# Autodesk Inventor assembly: 08-03-00-000_shifter_assembly
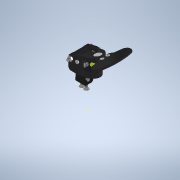
[picture p0: Inventor's stored thumbnail of the model, 180x180]
Saved by Autodesk Inventor 2020 (Build 240168000, 168)
## iProperties
Created: 2021-05-29
Part Number: 08-03-00-000_shifter_assembly
Document SubType Name: Assembly
Designer: Eric
Mass: 132.863 g
Surface Area: 203.28 cm^2
Volume: 20.5558 cm^3
Density: 6.46353 g/cm^3
Author: Eric
## Documents named in this file (15)
- C:\Users\Eric\Documents\repos\DIY_CAD_WheelButtonPlate\CAD\Inventor\08-05-00-000_shifter_assembly.iam
- C:\Users\Eric\Documents\repos\DIY_CAD_WheelButtonPlate\CAD\Inventor\08-05-01-002_shifter_base.ipt
- C:\Users\Eric\Documents\repos\DIY_CAD_WheelButtonPlate\CAD\Inventor\08-05-01-004_shifter_bottom.ipt
- C:\Users\Eric\Documents\repos\DIY_CAD_WheelButtonPlate\CAD\Inventor\08-05-01-003_shift_lever.ipt
- C:\Users\Eric\Documents\Inventor\Content Center Files\R2020\de-DE\DIN 7984\DIN 7984 - M3 x 8.ipt
- C:\Users\Eric\Documents\Inventor\Content Center Files\R2020\de-DE\DIN 7991(2)\DIN 7991 - M3x10.ipt
- C:\Users\Eric\Documents\Inventor\Content Center Files\R2020\de-DE\ISO 4035(1)\ISO 4035 - M3DIN EN.ipt
- C:\Users\Eric\Documents\repos\DIY_CAD_WheelButtonPlate\CAD\Inventor\08-05-01-005_shiftAndClutchHolder.ipt
- C:\Users\Eric\Documents\Inventor\Content Center Files\R2020\de-DE\DIN 7991(2)\DIN 7991 - M4x16.ipt
- C:\Users\Eric\Documents\Inventor\Content Center Files\R2020\de-DE\ISO 4032(1)\ISO 4032 - M4DIN EN.ipt
- C:\Users\Eric\Documents\repos\DIY_CAD_WheelButtonPlate\CAD\Inventor\08-05-02-006_Apem_yellow.ipt
- C:\Users\Eric\Documents\Inventor\Content Center Files\R2020\de-DE\ISO 4762(1)\DIN EN ISO 4762 - M4 x 40.ipt
- C:\Users\Eric\Documents\Inventor\Content Center Files\R2020\de-DE\ISO 4032(1)\ISO 4032 - M3DIN EN.ipt
- C:\Users\Eric\Documents\repos\DIY_CAD_WheelButtonPlate\CAD\Inventor\08-05-01-001_shifter_paddle.ipt
- C:\Users\Eric\Documents\repos\DIY_CAD_WheelButtonPlate\CAD\Inventor\08-04-02-004_magnet12x3.ipt
## Components (26 placed, 14 different names)
1. 08-05-01-002_shifter_base — Passend:5, Passend:16, Passend:17, Passend:18, Passend:26, Passend:27, Passend:29, Passend:31, Einfügen:5, Einfügen:6, Einfügen:9, Einfügen:10, Winkel:2, Winkel:3, Passend:38
2. 08-05-01-004_shifter_bottom — Passend:5, Passend:8, Winkel:1, Einfügen:7, Einfügen:8, Passend:36, Passend:37, Passend:39, Passend:40
3. 08-05-01-003_shift_lever — Passend:8, Passend:10, Passend:11, Fluchtend:2, Passend:13, Passend:15, Winkel:1, Passend:32, Passend:35, Passend:41, Passend:42
4. DIN 7984 M3 x 8:1 — Passend:31
5. DIN 7984 M3 x 8:2 — Passend:29, Passend:37, Passend:38
6. DIN 7991 M3x10:1 — Passend:11, Fluchtend:1, Fluchtend:2, Passend:12, Passend:34
7. DIN 7991 M3x10:2 — Passend:10, Fluchtend:1, Passend:14, Passend:33
8. DIN EN 24035 M3:1 — Passend:12, Passend:13
9. DIN EN 24035 M3:2 — Passend:14, Passend:15
10. 08-05-01-005_shiftAndClutchHolder:1 — Passend:16, Passend:17, Passend:18, Passend:19, Passend:20, Passend:21, Passend:22, Passend:23, Einfügen:3, Einfügen:4, Passend:24, Passend:25
11. DIN 7991 M4x16:1 — Passend:19
12. DIN 7991 M4x16:2 — Passend:20
13. DIN 7991 M4x16:3 — Passend:22, Fluchtend:3
14. DIN 7991 M4x16:4 — Passend:21, Fluchtend:3, Passend:23
15. DIN EN 24032 M4:1 — Einfügen:3, Passend:24
16. DIN EN 24032 M4:2 — Einfügen:4, Passend:25
17. 08-05-02-006_Apem_yellow:1 — Passend:26, Passend:27
18. DIN EN ISO 4762 M4 x 40:1 — Einfügen:5, Passend:35, Passend:36
19. DIN EN 24032 M4:3 — Einfügen:6
20. DIN EN 24032 M3:1 — Einfügen:7
21. DIN EN 24032 M3:2 — Einfügen:8
22. 08-05-01-001_shifter_paddle:1 — Passend:32, Passend:33, Passend:34
23. DIN EN 24032 M4:4 — Einfügen:9, Winkel:2
24. DIN EN 24032 M4:5 — Einfügen:10, Winkel:3
25. 08-04-02-004_magnet12x3:1 — Passend:39, Passend:40
26. 08-04-02-004_magnet12x3:2 — Passend:41, Passend:42
## Relationships (47: Mate 33, Insert 8, Flush 3, Angle 3)
- Passend:5 [Mate] (0.4 mm): 08-05-01-002_shifter_base ↔ 08-05-01-004_shifter_bottom
- Passend:8 [Mate] (0.2 mm): 08-05-01-004_shifter_bottom ↔ 08-05-01-003_shift_lever
- Passend:10 [Mate]: 08-05-01-003_shift_lever ↔ DIN 7991 M3x10:2
- Passend:11 [Mate]: 08-05-01-003_shift_lever ↔ DIN 7991 M3x10:1
- Fluchtend:1 [Flush]: DIN 7991 M3x10:1 ↔ DIN 7991 M3x10:2
- Fluchtend:2 [Flush] (-3.1 mm): 08-05-01-003_shift_lever ↔ DIN 7991 M3x10:1
- Passend:12 [Mate]: DIN 7991 M3x10:1 ↔ DIN EN 24035 M3:1
- Passend:13 [Mate]: 08-05-01-003_shift_lever ↔ DIN EN 24035 M3:1
- Passend:14 [Mate]: DIN 7991 M3x10:2 ↔ DIN EN 24035 M3:2
- Passend:15 [Mate]: 08-05-01-003_shift_lever ↔ DIN EN 24035 M3:2
- Passend:16 [Mate] (2 mm): 08-05-01-002_shifter_base ↔ 08-05-01-005_shiftAndClutchHolder:1
- Passend:17 [Mate]: 08-05-01-002_shifter_base ↔ 08-05-01-005_shiftAndClutchHolder:1
- Passend:18 [Mate]: 08-05-01-002_shifter_base ↔ 08-05-01-005_shiftAndClutchHolder:1
- Winkel:1 [Angle] (180 deg): 08-05-01-004_shifter_bottom ↔ 08-05-01-003_shift_lever
- Passend:19 [Mate]: 08-05-01-005_shiftAndClutchHolder:1 ↔ DIN 7991 M4x16:1
- Passend:20 [Mate]: 08-05-01-005_shiftAndClutchHolder:1 ↔ DIN 7991 M4x16:2
- Passend:21 [Mate]: 08-05-01-005_shiftAndClutchHolder:1 ↔ DIN 7991 M4x16:4
- Passend:22 [Mate]: 08-05-01-005_shiftAndClutchHolder:1 ↔ DIN 7991 M4x16:3
- Fluchtend:3 [Flush]: DIN 7991 M4x16:3 ↔ DIN 7991 M4x16:4
- Passend:23 [Mate] (-16.1 mm): 08-05-01-005_shiftAndClutchHolder:1 ↔ DIN 7991 M4x16:4
- Einfügen:3 [Insert]: 08-05-01-005_shiftAndClutchHolder:1 ↔ DIN EN 24032 M4:1
- Einfügen:4 [Insert]: 08-05-01-005_shiftAndClutchHolder:1 ↔ DIN EN 24032 M4:2
- Passend:24 [Mate]: 08-05-01-005_shiftAndClutchHolder:1 ↔ DIN EN 24032 M4:1
- Passend:25 [Mate]: 08-05-01-005_shiftAndClutchHolder:1 ↔ DIN EN 24032 M4:2
- Passend:26 [Mate]: 08-05-01-002_shifter_base ↔ 08-05-02-006_Apem_yellow:1
- Passend:27 [Mate]: 08-05-01-002_shifter_base ↔ 08-05-02-006_Apem_yellow:1
- Passend:29 [Mate]: 08-05-01-002_shifter_base ↔ DIN 7984 M3 x 8:2
- Passend:31 [Mate]: 08-05-01-002_shifter_base ↔ DIN 7984 M3 x 8:1
- Einfügen:5 [Insert]: 08-05-01-002_shifter_base ↔ DIN EN ISO 4762 M4 x 40:1
- Einfügen:6 [Insert]: 08-05-01-002_shifter_base ↔ DIN EN 24032 M4:3
- Einfügen:7 [Insert]: 08-05-01-004_shifter_bottom ↔ DIN EN 24032 M3:1
- Einfügen:8 [Insert]: 08-05-01-004_shifter_bottom ↔ DIN EN 24032 M3:2
- Passend:32 [Mate]: 08-05-01-003_shift_lever ↔ 08-05-01-001_shifter_paddle:1
- Passend:33 [Mate]: DIN 7991 M3x10:2 ↔ 08-05-01-001_shifter_paddle:1
- Passend:34 [Mate]: DIN 7991 M3x10:1 ↔ 08-05-01-001_shifter_paddle:1
- Passend:35 [Mate]: 08-05-01-003_shift_lever ↔ DIN EN ISO 4762 M4 x 40:1
- Passend:36 [Mate]: 08-05-01-004_shifter_bottom ↔ DIN EN ISO 4762 M4 x 40:1
- Passend:37 [Mate]: 08-05-01-004_shifter_bottom ↔ DIN 7984 M3 x 8:2
- Einfügen:9 [Insert]: 08-05-01-002_shifter_base ↔ DIN EN 24032 M4:4
- Einfügen:10 [Insert]: 08-05-01-002_shifter_base ↔ DIN EN 24032 M4:5
- Winkel:2 [Angle] (0 deg): 08-05-01-002_shifter_base ↔ DIN EN 24032 M4:4
- Winkel:3 [Angle] (0 deg): 08-05-01-002_shifter_base ↔ DIN EN 24032 M4:5
- Passend:38 [Mate]: 08-05-01-002_shifter_base ↔ DIN 7984 M3 x 8:2
- Passend:39 [Mate]: 08-05-01-004_shifter_bottom ↔ 08-04-02-004_magnet12x3:1
- Passend:40 [Mate]: 08-05-01-004_shifter_bottom ↔ 08-04-02-004_magnet12x3:1
- Passend:41 [Mate]: 08-05-01-003_shift_lever ↔ 08-04-02-004_magnet12x3:2
- Passend:42 [Mate]: 08-05-01-003_shift_lever ↔ 08-04-02-004_magnet12x3:2
